# Autodesk Inventor assembly: DPLX_A003_Lab_Version_Small_PV
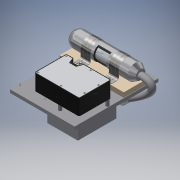
[picture p0: Inventor's stored thumbnail of the model, 180x180]
Saved by Autodesk Inventor 2018 (Build 220112000, 112)
## iProperties
Created: 2018-06-12
Part Number: DPLX_A003_Lab_Version_Small_PV
Document SubType Name: Assembly
Designer: DPLXuser
Author: DPLXuser
## Documents named in this file (11)
- C:\Users\DPLXuser\Documents\Michael Schwab\SPARK CAD Files\DPLX_A003_Lab_Version_Small_PV.iam
- C:\Users\DPLXuser\Documents\Michael Schwab\SPARK CAD Files\DPLX_P014_Lab_Baseplate_Small_PV.ipt
- C:\Users\DPLXuser\Documents\Michael Schwab\Aether PacknGo 6-4-18 8PM\RPi3.iam
- C:\Users\DPLXuser\Documents\Michael Schwab\Aether PacknGo 6-4-18 8PM\SSL Spark Gap with Insulation.iam
- C:\Users\DPLXuser\Documents\Michael Schwab\Aether PacknGo 6-4-18 8PM\SSL VIPE Insulated Mount.iam
- C:\Users\DPLXuser\Documents\Michael Schwab\Aether PacknGo 6-4-18 8PM\Ocean Optics Flame.iam
- C:\Users\DPLXuser\Documents\Michael Schwab\SPARK CAD Files\wire4.ipt
- C:\Users\DPLXuser\Documents\Michael Schwab\SPARK CAD Files\DPLX_P017_.5in _Standoff_smallplate.ipt
- C:\Users\DPLXuser\Documents\Michael Schwab\SPARK CAD Files\91771A085_18-8 SS FLAT HEAD PHILLIPS MACHINE SCREW.ipt
- C:\Users\DPLXuser\Documents\Michael Schwab\SPARK CAD Files\DPLX_P018_Crude_Battery_Placeholder_Smalltestmod.ipt
- C:\Users\DPLXuser\Documents\Michael Schwab\SPARK CAD Files\92000A107_18-8 SS METRIC PAN HEAD PHIL MACHINE SCREW.ipt
## Components (17 placed, 10 different names)
1. DPLX_P014_Lab_Baseplate_Small_PV:1 — Mate:1, Mate:2, Mate:4, Mate:7, Mate:8, Flush:1, Mate:9, Flush:10, Insert:1, Insert:2, Mate:23, Insert:3, Insert:4, Insert:5, Mate:24, Mate:25, Mate:26
2. RPi3:1 [sub-assembly] — Mate:9, Flush:10, Insert:6, Insert:7, Insert:8, Insert:9
3. SSL Spark Gap with Insulation:1 [sub-assembly] — Mate:1, Mate:2, Mate:4, Mate:14, Mate:15, Flush:7
4. SSL VIPE Insulated Mount:1 [sub-assembly] — Mate:7, Mate:8, Flush:1, Mate:13, Flush:6
5. Ocean Optics Flame:1 [sub-assembly]
6. wire4:1 — Flush:5, Flush:6, Flush:7
7. DPLX_P017_.5in _Standoff_smallplate:2 — Insert:2
8. DPLX_P017_.5in _Standoff_smallplate:3 — Insert:1
9. DPLX_P017_.5in _Standoff_smallplate:4 — Mate:23
10. 91771A085_18-8 SS FLAT HEAD PHILLIPS MACHINE SCREW:1 — Insert:4
11. 91771A085_18-8 SS FLAT HEAD PHILLIPS MACHINE SCREW:2 — Insert:3
12. 91771A085_18-8 SS FLAT HEAD PHILLIPS MACHINE SCREW:3 — Insert:5
13. DPLX_P018_Crude_Battery_Placeholder_Smalltestmod:1 — Mate:24, Mate:25, Mate:26
14. 92000A107_18-8 SS METRIC PAN HEAD PHIL MACHINE SCREW:1 — Insert:6
15. 92000A107_18-8 SS METRIC PAN HEAD PHIL MACHINE SCREW:2 — Insert:9
16. 92000A107_18-8 SS METRIC PAN HEAD PHIL MACHINE SCREW:3 — Insert:8
17. 92000A107_18-8 SS METRIC PAN HEAD PHIL MACHINE SCREW:4 — Insert:7
## Relationships (27: Mate 13, Insert 9, Flush 5)
- Mate:1: DPLX_P014_Lab_Baseplate_Small_PV:1 ↔ SSL Spark Gap with Insulation:1
- Mate:2: DPLX_P014_Lab_Baseplate_Small_PV:1 ↔ SSL Spark Gap with Insulation:1
- Mate:4: DPLX_P014_Lab_Baseplate_Small_PV:1 ↔ SSL Spark Gap with Insulation:1
- Mate:7: DPLX_P014_Lab_Baseplate_Small_PV:1 ↔ SSL VIPE Insulated Mount:1
- Mate:8: DPLX_P014_Lab_Baseplate_Small_PV:1 ↔ SSL VIPE Insulated Mount:1
- Flush:1 (31.75 mm): DPLX_P014_Lab_Baseplate_Small_PV:1 ↔ SSL VIPE Insulated Mount:1
- Mate:9: DPLX_P014_Lab_Baseplate_Small_PV:1 ↔ RPi3:1
- Mate:13: SSL VIPE Insulated Mount:1
- Mate:14: SSL Spark Gap with Insulation:1
- Mate:15: SSL Spark Gap with Insulation:1
- Flush:5: wire4:1
- Flush:6: SSL VIPE Insulated Mount:1 ↔ wire4:1
- Flush:7: SSL Spark Gap with Insulation:1 ↔ wire4:1
- Flush:10 (12.7 mm): DPLX_P014_Lab_Baseplate_Small_PV:1 ↔ RPi3:1
- Insert:1: DPLX_P014_Lab_Baseplate_Small_PV:1 ↔ DPLX_P017_.5in _Standoff_smallplate:3
- Insert:2: DPLX_P014_Lab_Baseplate_Small_PV:1 ↔ DPLX_P017_.5in _Standoff_smallplate:2
- Mate:23: DPLX_P014_Lab_Baseplate_Small_PV:1 ↔ DPLX_P017_.5in _Standoff_smallplate:4
- Insert:3: DPLX_P014_Lab_Baseplate_Small_PV:1 ↔ 91771A085_18-8 SS FLAT HEAD PHILLIPS MACHINE SCREW:2
- Insert:4: DPLX_P014_Lab_Baseplate_Small_PV:1 ↔ 91771A085_18-8 SS FLAT HEAD PHILLIPS MACHINE SCREW:1
- Insert:5: DPLX_P014_Lab_Baseplate_Small_PV:1 ↔ 91771A085_18-8 SS FLAT HEAD PHILLIPS MACHINE SCREW:3
- Mate:24: DPLX_P014_Lab_Baseplate_Small_PV:1 ↔ DPLX_P018_Crude_Battery_Placeholder_Smalltestmod:1
- Mate:25: DPLX_P014_Lab_Baseplate_Small_PV:1 ↔ DPLX_P018_Crude_Battery_Placeholder_Smalltestmod:1
- Mate:26 (6.3246 mm): DPLX_P014_Lab_Baseplate_Small_PV:1 ↔ DPLX_P018_Crude_Battery_Placeholder_Smalltestmod:1
- Insert:6: RPi3:1 ↔ 92000A107_18-8 SS METRIC PAN HEAD PHIL MACHINE SCREW:1
- Insert:7: RPi3:1 ↔ 92000A107_18-8 SS METRIC PAN HEAD PHIL MACHINE SCREW:4
- Insert:8: RPi3:1 ↔ 92000A107_18-8 SS METRIC PAN HEAD PHIL MACHINE SCREW:3
- Insert:9: RPi3:1 ↔ 92000A107_18-8 SS METRIC PAN HEAD PHIL MACHINE SCREW:2
